# Autodesk Inventor assembly: Joining Plate for 4040 Assembly - A
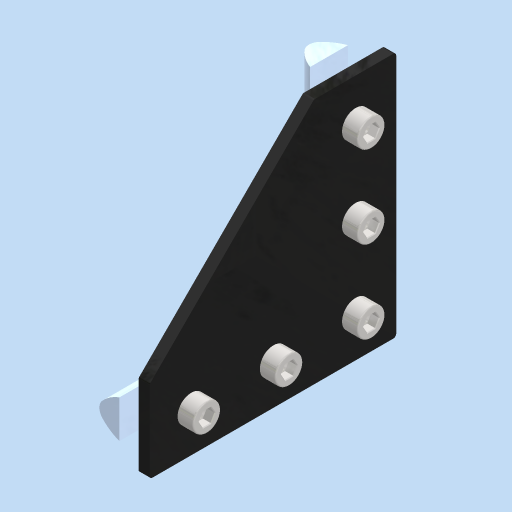
[picture p0: Inventor's stored thumbnail of the model, 512x512]
Saved by Autodesk Inventor 2023.2 (Build 272271000, 271)
## iProperties
Created: 2023-11-20
Part Number: Joining Plate for 4040 Assembly - A
Document SubType Name: Assembly
Designer: Nils Bade
Author: Nils Bade
## Documents named in this file (6)
- C:\Users\nilsb\Documents\Inventor\Projektarbeit-Bade\RatRig_modified\Joining Plate for 4040 Assembly - A - Kopie.iam
- Joining Plate for 4040 Assembly - A - ItemNuts.iam
- C:\Users\nilsb\Documents\Inventor\Projektarbeit-Bade\RatRig_Standards\Joining Plate for 3030 - 90 Degree - Black Anodized v2.ipt
- C:\Users\nilsb\Documents\Inventor\Projektarbeit-Bade\Schrauben\Cap Head Screw M6x12 v2.ipt
- C:\Users\nilsb\Documents\Inventor\Projektarbeit-Bade\ITEM\item_Nutenstein 8 - M6_0002623.ipt
- item_Nutenstein 8 - M6_0002623.ipt
## Components (11 placed, 3 different names)
1. Joining Plate for 3030 - 90 Degree - Black Anodized v2:2 — Passend:1, Passend:2, Passend:3, Passend:4, Passend:5, Passend:6, Passend:7, Passend:8, Passend:9, Passend:10, Winkel:1, Winkel:2, Winkel:3, Winkel:4, Winkel:5, Passend:16, Passend:17, Passend:18, Passend:19, Passend:20
2. Cap Head Screw M6x12 v2:1 — Passend:5, Passend:6, Passend:13
3. Cap Head Screw M6x12 v2:2 — Passend:4, Passend:7, Passend:12
4. Cap Head Screw M6x12 v2:3 — Passend:2, Passend:9, Passend:14
5. Cap Head Screw M6x12 v2:4 — Passend:3, Passend:10, Passend:15
6. Cap Head Screw M6x12 v2:5 — Passend:1, Passend:8, Passend:11
7. item_Nutenstein 8 - M6_0002623:1 — Passend:13, Winkel:3, Passend:20
8. item_Nutenstein 8 - M6_0002623:2 — Passend:12, Winkel:2, Passend:19
9. item_Nutenstein 8 - M6_0002623:3 — Passend:11, Winkel:1, Passend:18
10. item_Nutenstein 8 - M6_0002623:4 — Passend:14, Winkel:4, Passend:17
11. item_Nutenstein 8 - M6_0002623:5 — Passend:15, Winkel:5, Passend:16
## Relationships (25: Mate 20, Angle 5)
- Passend:1 [Mate]: Joining Plate for 3030 - 90 Degree - Black Anodized v2:2 ↔ Cap Head Screw M6x12 v2:5
- Passend:2 [Mate]: Joining Plate for 3030 - 90 Degree - Black Anodized v2:2 ↔ Cap Head Screw M6x12 v2:3
- Passend:3 [Mate]: Joining Plate for 3030 - 90 Degree - Black Anodized v2:2 ↔ Cap Head Screw M6x12 v2:4
- Passend:4 [Mate]: Joining Plate for 3030 - 90 Degree - Black Anodized v2:2 ↔ Cap Head Screw M6x12 v2:2
- Passend:5 [Mate]: Joining Plate for 3030 - 90 Degree - Black Anodized v2:2 ↔ Cap Head Screw M6x12 v2:1
- Passend:6 [Mate]: Joining Plate for 3030 - 90 Degree - Black Anodized v2:2 ↔ Cap Head Screw M6x12 v2:1
- Passend:7 [Mate]: Joining Plate for 3030 - 90 Degree - Black Anodized v2:2 ↔ Cap Head Screw M6x12 v2:2
- Passend:8 [Mate]: Joining Plate for 3030 - 90 Degree - Black Anodized v2:2 ↔ Cap Head Screw M6x12 v2:5
- Passend:9 [Mate]: Joining Plate for 3030 - 90 Degree - Black Anodized v2:2 ↔ Cap Head Screw M6x12 v2:3
- Passend:10 [Mate]: Joining Plate for 3030 - 90 Degree - Black Anodized v2:2 ↔ Cap Head Screw M6x12 v2:4
- Passend:11 [Mate]: Cap Head Screw M6x12 v2:5 ↔ item_Nutenstein 8 - M6_0002623:3
- Passend:12 [Mate]: Cap Head Screw M6x12 v2:2 ↔ item_Nutenstein 8 - M6_0002623:2
- Passend:13 [Mate]: Cap Head Screw M6x12 v2:1 ↔ item_Nutenstein 8 - M6_0002623:1
- Passend:14 [Mate]: Cap Head Screw M6x12 v2:3 ↔ item_Nutenstein 8 - M6_0002623:4
- Passend:15 [Mate]: Cap Head Screw M6x12 v2:4 ↔ item_Nutenstein 8 - M6_0002623:5
- Winkel:1 [Angle] (0 deg): Joining Plate for 3030 - 90 Degree - Black Anodized v2:2 ↔ item_Nutenstein 8 - M6_0002623:3
- Winkel:2 [Angle] (0 deg): Joining Plate for 3030 - 90 Degree - Black Anodized v2:2 ↔ item_Nutenstein 8 - M6_0002623:2
- Winkel:3 [Angle] (0 deg): Joining Plate for 3030 - 90 Degree - Black Anodized v2:2 ↔ item_Nutenstein 8 - M6_0002623:1
- Winkel:4 [Angle] (0 deg): Joining Plate for 3030 - 90 Degree - Black Anodized v2:2 ↔ item_Nutenstein 8 - M6_0002623:4
- Winkel:5 [Angle] (0 deg): Joining Plate for 3030 - 90 Degree - Black Anodized v2:2 ↔ item_Nutenstein 8 - M6_0002623:5
- Passend:16 [Mate] (5.5 mm): Joining Plate for 3030 - 90 Degree - Black Anodized v2:2 ↔ item_Nutenstein 8 - M6_0002623:5
- Passend:17 [Mate] (5.5 mm): Joining Plate for 3030 - 90 Degree - Black Anodized v2:2 ↔ item_Nutenstein 8 - M6_0002623:4
- Passend:18 [Mate] (5.5 mm): Joining Plate for 3030 - 90 Degree - Black Anodized v2:2 ↔ item_Nutenstein 8 - M6_0002623:3
- Passend:19 [Mate] (5.5 mm): Joining Plate for 3030 - 90 Degree - Black Anodized v2:2 ↔ item_Nutenstein 8 - M6_0002623:2
- Passend:20 [Mate] (5.5 mm): Joining Plate for 3030 - 90 Degree - Black Anodized v2:2 ↔ item_Nutenstein 8 - M6_0002623:1
